# Autodesk Inventor assembly: søjle+top
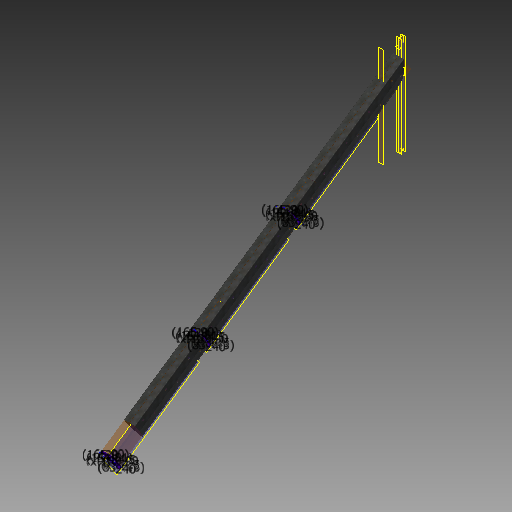
[picture p0: Inventor's stored thumbnail of the model, 512x512]
Saved by Autodesk Inventor 2018 (Build 220112000, 112)
## iProperties
Created: 2019-09-25
Part Number: søjle+top
Document SubType Name: Assembly
Designer: gust3763
Author: gust3763
## Documents named in this file (4)
- H:\INVENTOR 2018\WF_navn_2018\DESIGNS\H4\trappe\søjle+top.iam
- H:\INVENTOR 2018\WF_navn_2018\DESIGNS\H4\trappe\modul top.iam
- H:\INVENTOR 2018\WF_navn_2018\DESIGNS\H4\trappe\søjle\stilladssøjle.iam
- H:\INVENTOR 2018\WF_navn_2018\DESIGNS\H4\trappe\modul.iam
## Components (4 placed, 3 different names)
1. stilladssøjle:2 [sub-assembly] — Mate:3, Mate:4, øre
2. modul top:1 [sub-assembly] — Mate:3, Mate:4, øre, Flush:1, Flush:3, Mate:6
3. modul:1 [sub-assembly] — Flush:1, Flush:2, Flush:3, Flush:4, Mate:6, Mate:7
4. modul:2 [sub-assembly] — Flush:2, Flush:4, Mate:7
## Relationships (10: Mate 6, Flush 4)
- [Mate]: stilladssøjle:2 ↔ modul top:1
- Mate:3: stilladssøjle:2 ↔ modul top:1
- Mate:4: stilladssøjle:2 ↔ modul top:1
- øre [Mate]: stilladssøjle:2 ↔ modul top:1
- Flush:1: modul top:1 ↔ modul:1
- Flush:2: modul:1 ↔ modul:2
- Flush:3: modul top:1 ↔ modul:1
- Flush:4: modul:1 ↔ modul:2
- Mate:6 (2 mm): modul top:1 ↔ modul:1
- Mate:7 (2 mm): modul:1 ↔ modul:2
